# Autodesk Inventor assembly: Robot Assembly
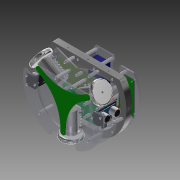
[picture p0: Inventor's stored thumbnail of the model, 180x180]
Saved by Autodesk Inventor 2015 (Build 190159000, 159)
## iProperties
Created: 2016-02-17
Part Number: Robot Assembly
Document SubType Name: Assembly
Designer: 23902
Author: 23902
## Documents named in this file (31)
- C:\Users\James Yelland\git\Work\Design\3D Printing\Version 4\Robot Assembly.iam
- C:\Users\James Yelland\git\Work\Design\3D Printing\Version 4\Motor Mount Plate.ipt
- C:\Users\James Yelland\git\Work\Design\3D Printing\Motor Mount Bracket.ipt
- C:\Users\James Yelland\git\Work\Design\3D Printing\Motor.ipt
- C:\Users\James Yelland\git\Work\Design\3D Printing\Wheel.ipt
- C:\Users\James Yelland\git\Work\Design\3D Printing\Version 4\Middle Plate.ipt
- C:\Users\James Yelland\git\Work\Design\3D Printing\Version 4\Standoff 20.ipt
- C:\Users\James Yelland\git\Work\Design\3D Printing\Version 4\Light Sensor Plate.ipt
- C:\Users\James Yelland\git\Work\Design\3D Printing\Version 4\Light Sensor PCB.ipt
- C:\Users\James Yelland\git\Work\Design\3D Printing\Version 4\Standoff 10.ipt
- C:\Users\James Yelland\git\Work\Design\3D Printing\ArduinoMEGA2560.ipt
- C:\Users\James Yelland\git\Work\Design\3D Printing\Version 4\Standoff 30.ipt
- C:\Users\James Yelland\git\Work\Design\3D Printing\Version 4\Veroboard.ipt
- C:\Users\James Yelland\git\Work\Design\3D Printing\Version 4\M3x20 Screw Nylon.ipt
- C:\Users\James Yelland\git\Work\Design\3D Printing\Version 4\M3x10 Screw Nylon.ipt
- C:\Users\James Yelland\git\Work\Design\3D Printing\Version 4\M3x6 Screw Nylon.ipt
- C:\Users\James Yelland\git\Work\Design\3D Printing\Version 4\M3 Nut Nylon.ipt
- C:\Users\James Yelland\git\Work\Design\3D Printing\Version 4\M3x10 Screw Steel.ipt
- C:\Users\James Yelland\git\Work\Design\3D Printing\Version 4\M3 Nut Steel.ipt
- C:\Users\James Yelland\git\Work\Design\3D Printing\HC-SR04 Sonar.ipt
- C:\Users\James Yelland\git\Work\Design\3D Printing\Version 4\Sonar Mount.ipt
- C:\Users\James Yelland\git\Work\Design\3D Printing\Version 4\M2x10 Screw Steel.ipt
- C:\Users\James Yelland\git\Work\Design\3D Printing\Version 4\M2 Nut Steel.ipt
- C:\Users\James Yelland\git\Work\Design\3D Printing\lcd05-16x2.ipt
- C:\Users\James Yelland\git\Work\Design\3D Printing\Version 4\LCD Plate.ipt
- C:\Users\James Yelland\git\Work\Design\3D Printing\Version 4\Top Plate.ipt
- C:\Users\James Yelland\git\Work\Design\3D Printing\Version 4\Battery.ipt
- C:\Users\James Yelland\git\Work\Design\3D Printing\Version 4\Switch Nut.ipt
- C:\Users\James Yelland\git\Work\Design\3D Printing\Version 4\Switch.ipt
- C:\Users\James Yelland\git\Work\Design\3D Printing\Version 4\Standoff 40.ipt
- C:\Users\James Yelland\git\Work\Design\3D Printing\Compass.ipt
## Components (161 placed, 30 different names)
1. Motor Mount Plate:1 — Mate:1, Mate:2, Mate:3, Mate:22, Mate:23, Mate:24, Mate:25, Mate:26, Mate:27, Mate:28, Mate:29, Mate:30, Mate:31, Mate:32, Mate:33, Mate:34, Mate:35, Mate:101, Mate:102, Mate:103, Mate:104, Mate:113, Mate:114, Mate:115, Mate:116, Mate:117, Mate:118, Mate:127, Mate:128, Mate:129, Mate:130, Mate:131, Mate:132, Mate:155, Mate:156, Mate:157, Mate:158, Mate:159, Mate:160, Mate:161, Mate:162, Mate:182, Mate:183, Mate:184, Mate:185, Mate:186, Mate:187, Mate:203, Mate:204, Mate:205, Mate:206, Mate:207, Mate:208, Mate:209, Mate:210, Mate:211, Mate:212, Mate:213, Mate:214, Mate:223, Mate:224, Mate:225, Mate:226, Mate:227, Mate:228, Mate:229, Mate:230, Mate:249, Mate:250, Mate:251, Mate:252, Mate:253, Mate:254, Mate:255, Mate:256, Mate:257, Mate:269, Mate:270, Mate:272, Mate:274, Mate:278, Mate:280, Mate:281, Mate:282, Mate:284, Mate:288, Mate:289, Mate:290, Mate:291, Mate:293, Mate:294, Mate:295, Mate:296, Mate:297, Mate:298, Mate:299, Mate:300, Mate:301, Mate:302, Mate:303
2. Motor Mount Bracket:1 — Mate:1, Mate:11, Mate:14, Mate:15, Mate:24, Mate:25, Mate:275, Mate:276, Mate:286, Mate:287
3. Motor:1 — Mate:10, Mate:16, Mate:17, Mate:21, Flush:3
4. Wheel:1 — Mate:19, Flush:1
5. Motor Mount Bracket:2 — Mate:2, Mate:10, Mate:16, Mate:17, Mate:22, Mate:23, Mate:267, Mate:268, Mate:277, Mate:279
6. Motor:2 — Mate:11, Mate:14, Mate:15, Mate:19, Flush:1
7. Wheel:2 — Mate:20, Flush:2
8. Motor Mount Bracket:3 — Mate:3, Mate:12, Mate:13, Mate:18, Mate:26, Mate:27, Mate:271, Mate:273, Mate:283, Mate:285
9. Motor:3 — Mate:12, Mate:13, Mate:18, Mate:20, Flush:2
10. Wheel:3 — Mate:21, Flush:3
11. Middle Plate:1 — Mate:36, Mate:37, Mate:38, Mate:191, Mate:192, Mate:193, Mate:194, Mate:195, Mate:196, Mate:197, Mate:198, Mate:199, Mate:200, Mate:201, Mate:202, Mate:315, Mate:316, Mate:317, Mate:318, Mate:319, Mate:320, Mate:321, Mate:322, Mate:323, Mate:324, Mate:325, Mate:326, Mate:327, Mate:328, Mate:329, Mate:330, Mate:452, Mate:453, Mate:454, Mate:455, Mate:462, Mate:463, Mate:464, Mate:465
12. Standoff 20:1 — Mate:28, Mate:33, Mate:38
13. Standoff 20:2 — Mate:29, Mate:35, Mate:36
14. Standoff 20:3 — Mate:31, Mate:32
15. Standoff 20:4 — Mate:30, Mate:34, Mate:37
16. Light Sensor Plate:1 — Mate:152, Mate:153, Mate:154, Mate:163, Mate:164, Mate:165, Mate:215, Mate:216, Mate:217, Mate:218, Mate:219, Mate:220, Mate:221, Mate:222, Mate:362, Mate:384, Mate:385, Mate:386, Mate:387, Mate:388, Mate:389, Mate:390, Mate:391, Mate:392, Mate:393, Mate:394, Mate:395, Mate:396, Mate:510, Mate:511, Mate:512, Mate:515
17. Light Sensor PCB:1 — Mate:152, Mate:153, Mate:154
18. Standoff 20:5 — Mate:103, Mate:104
19. Standoff 20:6 — Mate:101, Mate:102
20. Standoff 10:1 — Mate:114, Mate:128, Mate:263
21. Standoff 10:2 — Mate:115, Mate:129, Mate:266
22. Standoff 10:3 — Mate:116, Mate:130, Mate:133, Mate:260
23. Standoff 10:4 — Mate:118, Mate:131, Mate:259
24. Standoff 10:5 — Mate:117, Mate:126, Mate:132, Mate:261
25. Standoff 10:6 — Mate:113, Mate:125, Mate:127, Mate:265
26. -  -:1 — Mate:125, Mate:126, Mate:133, Mate:234, Mate:235, Mate:236, Mate:237, Mate:238, Mate:239, Mate:240, Mate:241, Mate:242, Mate:243, Mate:244, Mate:245
27. Standoff 30:1 — Mate:157, Mate:162
28. Standoff 30:2 — Mate:159, Mate:161
29. Standoff 30:3 — Mate:155, Mate:156, Mate:163, Mate:164
30. Standoff 30:4 — Mate:158, Mate:160, Mate:165
31. Standoff 10:7 — Mate:182, Mate:186, Mate:190, Mate:258
32. Standoff 10:8 — Mate:183, Mate:187, Mate:188, Mate:189, Mate:262
33. Standoff 10:9 — Mate:184, Mate:185, Mate:264
34. Veroboard:1 — Mate:188, Mate:189, Mate:190, Mate:231, Mate:232, Mate:233, Mate:246, Mate:247, Mate:248
35. M3x20 Screw Nylon:1 — Mate:192, Mate:201
36. M3x20 Screw Nylon:2 — Mate:193, Mate:202
37. M3x20 Screw Nylon:3 — Mate:194, Mate:199
38. M3x20 Screw Nylon:4 — Mate:195, Mate:198
39. M3x20 Screw Nylon:5 — Mate:196, Mate:197
40. M3x20 Screw Nylon:6 — Mate:191, Mate:200
41. M3x10 Screw Nylon:1 — Mate:208, Mate:209
42. M3x10 Screw Nylon:2 — Mate:207, Mate:210
43. M3x10 Screw Nylon:3 — Mate:206, Mate:211
44. M3x10 Screw Nylon:4 — Mate:205, Mate:212
45. M3x10 Screw Nylon:5 — Mate:204, Mate:213
46. M3x10 Screw Nylon:6 — Mate:203, Mate:214
47. M3x10 Screw Nylon:7 — Mate:215, Mate:219
48. M3x10 Screw Nylon:8 — Mate:216, Mate:220
49. M3x10 Screw Nylon:9 — Mate:224, Mate:225
50. M3x10 Screw Nylon:10 — Mate:218, Mate:222
51. M3x10 Screw Nylon:11 — Mate:217, Mate:221
52. M3x10 Screw Nylon:12 — Mate:228, Mate:229
53. M3x10 Screw Nylon:13 — Mate:227, Mate:230
54. M3x10 Screw Nylon:14 — Mate:223, Mate:226
55. M3x6 Screw Nylon:1 — Mate:231, Mate:246
56. M3x6 Screw Nylon:2 — Mate:235, Mate:240
57. M3x6 Screw Nylon:3 — Mate:236, Mate:242
58. M3x6 Screw Nylon:4 — Mate:237, Mate:245
59. M3x6 Screw Nylon:5 — Mate:239, Mate:244
60. M3x6 Screw Nylon:6 — Mate:238, Mate:241
61. M3x6 Screw Nylon:7 — Mate:232, Mate:247
62. M3x6 Screw Nylon:8 — Mate:234, Mate:243
63. M3x6 Screw Nylon:9 — Mate:233, Mate:248
64. M3 Nut Nylon:1 — Mate:253, Mate:260
65. M3 Nut Nylon:2 — Mate:252, Mate:258
66. M3 Nut Nylon:3 — Mate:254, Mate:262
67. M3 Nut Nylon:4 — Mate:255, Mate:261
68. M3 Nut Nylon:5 — Mate:257, Mate:266
69. M3 Nut Nylon:6 — Mate:256, Mate:264
70. M3 Nut Nylon:7 — Mate:251, Mate:259
71. M3 Nut Nylon:8 — Mate:250, Mate:265
72. M3 Nut Nylon:9 — Mate:249, Mate:263
73. M3x10 Screw Steel:1 — Mate:271, Mate:272, Mate:292
74. M3x10 Screw Steel:2 — Mate:273, Mate:274, Mate:310
75. M3x10 Screw Steel:3 — Mate:268, Mate:269, Mate:307
76. M3x10 Screw Steel:4 — Mate:267, Mate:270, Mate:306
77. M3x10 Screw Steel:5 — Mate:283, Mate:284, Mate:308
78. M3x10 Screw Steel:6 — Mate:279, Mate:280, Mate:304
79. M3x10 Screw Steel:7 — Mate:277, Mate:278, Mate:305
80. M3x10 Screw Steel:8 — Mate:275, Mate:282, Mate:311
81. M3x10 Screw Steel:9 — Mate:287, Mate:288, Mate:314
82. M3x10 Screw Steel:10 — Mate:286, Mate:289, Mate:312
83. M3x10 Screw Steel:11 — Mate:285, Mate:290, Mate:309
84. M3x10 Screw Steel:12 — Mate:276, Mate:281, Mate:313
85. M3 Nut Steel:1 — Mate:295, Mate:314
86. M3 Nut Steel:2 — Mate:291, Mate:292
87. M3 Nut Steel:3 — Mate:294, Mate:312
88. M3 Nut Steel:4 — Mate:296, Mate:311
89. M3 Nut Steel:5 — Mate:298, Mate:310
90. M3 Nut Steel:6 — Mate:297, Mate:304
91. M3 Nut Steel:7 — Mate:300, Mate:305
92. M3 Nut Steel:8 — Mate:299, Mate:308
93. M3 Nut Steel:9 — Mate:301, Mate:306
94. M3 Nut Steel:10 — Mate:302, Mate:309
95. M3 Nut Steel:11 — Mate:293, Mate:313
96. M3 Nut Steel:12 — Mate:303, Mate:307
97. Standoff 30:5 — Mate:315, Mate:321
98. Standoff 30:6 — Mate:316, Mate:322
99. Standoff 30:7 — Mate:317, Mate:320, Mate:473, Mate:474
100. Standoff 30:8 — Mate:318, Mate:319, Mate:475
101. M3x20 Screw Nylon:7 — Mate:323, Mate:330
102. M3x20 Screw Nylon:8 — Mate:326, Mate:328
103. M3x20 Screw Nylon:9 — Mate:325, Mate:327
104. M3x20 Screw Nylon:10 — Mate:324, Mate:329
105. HC-SR04 Sonar:1 — Mate:360, Mate:376, Mate:377, Mate:380, Mate:381
106. Sonar Mount:1 — Mate:360, Mate:361, Mate:362, Mate:384, Mate:385, Mate:408, Mate:410, Mate:383, Mate:508, Mate:516
107. M2x10 Screw Steel:1 — Mate:376, Mate:377, Mate:379, Mate:361
108. M2 Nut Steel:1 — Mate:379
109. M2 Nut Steel:2 — Mate:508, Mate:509
110. M2x10 Screw Steel:2 — Mate:380, Mate:381, Mate:383, Mate:509
111. HC-SR04 Sonar:2 — Mate:397, Mate:398, Mate:399, Mate:400, Mate:401, Mate:404, Mate:405
112. Sonar Mount:2 — Mate:386, Mate:387, Mate:388, Mate:397, Mate:398, Mate:399, Mate:402, Mate:403, Mate:412, Mate:414, Mate:513
113. M3x10 Screw Nylon:24 — Mate:394, Mate:396, Mate:409
114. M3x10 Screw Nylon:25 — Mate:393, Mate:395, Mate:411
115. M3x10 Screw Nylon:26 — Mate:389, Mate:390, Mate:413
116. M3x10 Screw Nylon:27 — Mate:391, Mate:392, Mate:415
117. M2 Nut Steel:3 — Mate:403, Mate:406
118. M2x10 Screw Steel:3 — Mate:400, Mate:404, Mate:407
119. M2 Nut Steel:4 — Mate:402, Mate:407
120. M2x10 Screw Steel:4 — Mate:401, Mate:405, Mate:406
121. M3 Nut Nylon:10 — Mate:408, Mate:409
122. M3 Nut Nylon:11 — Mate:410, Mate:411
123. M3 Nut Nylon:12 — Mate:414, Mate:415
124. M3 Nut Nylon:13 — Mate:412, Mate:413
125. Standoff 20:7 — Mate:453, Mate:454, Mate:456, Mate:457
126. Standoff 20:8 — Mate:452, Mate:455, Mate:458
127. LCD Plate:1 — Mate:456, Mate:457, Mate:458, Mate:466, Mate:467, Mate:468, Mate:469, Mate:470, Mate:471, Mate:472, Mate:518, Mate:519, Mate:520, Mate:521, Mate:522, Mate:523, Mate:524, Mate:525
128. M3x20 Screw Nylon:11 — Mate:462, Mate:463
129. M3x20 Screw Nylon:12 — Mate:464, Mate:465
130. M3x10 Screw Nylon:36 — Mate:468, Mate:469
131. M3x10 Screw Nylon:37 — Mate:466, Mate:467
132. lcd05-16x2:1 — Mate:470, Mate:471, Mate:472, Mate:526, Mate:527, Mate:528, Mate:529
133. Top Plate:1 — Mate:473, Mate:474, Mate:475, Mate:476, Mate:477, Mate:478, Mate:479, Mate:480, Mate:481, Mate:482, Mate:483, Mate:484, Mate:485, Mate:486, Mate:487, Mate:488, Mate:489, Mate:490, Mate:491, Mate:492, Mate:493, Mate:494, Mate:495, Flush:4, Flush:5, Mate:496, Mate:497, Mate:507, Flush:6, Flush:7
134. M3x10 Screw Nylon:38 — Mate:489, Mate:491
135. M3x10 Screw Nylon:39 — Mate:503, Mate:504
136. M3x10 Screw Nylon:40 — Mate:488, Mate:490
137. M3x10 Screw Nylon:41 — Mate:505, Mate:506
138. Battery:1 — Mate:507, Flush:6, Flush:7
139. Switch Nut:1 — Mate:496, Mate:499
140. Switch:1 — Mate:492, Mate:495, Flush:5, Mate:499
141. Switch Nut:2 — Mate:497, Mate:498
142. Switch:2 — Mate:493, Mate:494, Flush:4, Mate:498
143. Standoff 40:1 — Mate:477, Mate:487, Mate:500, Mate:501
144. Standoff 40:2 — Mate:476, Mate:486, Mate:502
145. M3x10 Screw Nylon:42 — Mate:480, Mate:482
146. M3x10 Screw Nylon:43 — Mate:478, Mate:484
147. M3x10 Screw Nylon:44 — Mate:481, Mate:483
148. M3x10 Screw Nylon:45 — Mate:479, Mate:485
149. Compass:1 — Mate:500, Mate:501, Mate:502, Mate:503, Mate:504, Mate:505, Mate:506
150. M3x10 Screw Nylon:46 — Mate:511, Mate:515, Mate:517
151. M3x10 Screw Nylon:47 — Mate:510, Mate:512, Mate:514
152. M3 Nut Steel:14 — Mate:513, Mate:514
153. M3 Nut Nylon:14 — Mate:516, Mate:517
154. M2x10 Screw Steel:5 — Mate:524, Mate:525, Mate:530
155. M2x10 Screw Steel:6 — Mate:522, Mate:523, Mate:533
156. M2x10 Screw Steel:7 — Mate:520, Mate:521, Mate:532
157. M2x10 Screw Steel:8 — Mate:518, Mate:519, Mate:531
158. M2 Nut Steel:5 — Mate:529, Mate:533
159. M2 Nut Steel:6 — Mate:528, Mate:532
160. M2 Nut Steel:7 — Mate:527, Mate:531
161. M2 Nut Steel:8 — Mate:526, Mate:530
## Relationships (341: Mate 334, Flush 7)
- Mate:1: Motor Mount Plate:1 ↔ Motor Mount Bracket:1
- Mate:2: Motor Mount Plate:1 ↔ Motor Mount Bracket:2
- Mate:3: Motor Mount Plate:1 ↔ Motor Mount Bracket:3
- Mate:10: Motor:1 ↔ Motor Mount Bracket:2
- Mate:11: Motor Mount Bracket:1 ↔ Motor:2
- Mate:12: Motor Mount Bracket:3 ↔ Motor:3
- Mate:13: Motor Mount Bracket:3 ↔ Motor:3
- Mate:14: Motor Mount Bracket:1 ↔ Motor:2
- Mate:15: Motor Mount Bracket:1 ↔ Motor:2
- Mate:16: Motor:1 ↔ Motor Mount Bracket:2
- Mate:17: Motor:1 ↔ Motor Mount Bracket:2
- Mate:18: Motor Mount Bracket:3 ↔ Motor:3
- Mate:19: Wheel:1 ↔ Motor:2
- Flush:1: Wheel:1 ↔ Motor:2
- Mate:20: Wheel:2 ↔ Motor:3
- Flush:2: Wheel:2 ↔ Motor:3
- Mate:21: Motor:1 ↔ Wheel:3
- Flush:3: Motor:1 ↔ Wheel:3
- Mate:22: Motor Mount Plate:1 ↔ Motor Mount Bracket:2
- Mate:23: Motor Mount Plate:1 ↔ Motor Mount Bracket:2
- Mate:24: Motor Mount Plate:1 ↔ Motor Mount Bracket:1
- Mate:25: Motor Mount Plate:1 ↔ Motor Mount Bracket:1
- Mate:26: Motor Mount Plate:1 ↔ Motor Mount Bracket:3
- Mate:27: Motor Mount Plate:1 ↔ Motor Mount Bracket:3
- Mate:28: Motor Mount Plate:1 ↔ Standoff 20:1
- Mate:29: Motor Mount Plate:1 ↔ Standoff 20:2
- Mate:30: Motor Mount Plate:1 ↔ Standoff 20:4
- Mate:31: Motor Mount Plate:1 ↔ Standoff 20:3
- Mate:32: Motor Mount Plate:1 ↔ Standoff 20:3
- Mate:33: Motor Mount Plate:1 ↔ Standoff 20:1
- Mate:34: Motor Mount Plate:1 ↔ Standoff 20:4
- Mate:35: Motor Mount Plate:1 ↔ Standoff 20:2
- Mate:36: Middle Plate:1 ↔ Standoff 20:2
- Mate:37: Middle Plate:1 ↔ Standoff 20:4
- Mate:38: Middle Plate:1 ↔ Standoff 20:1
- Mate:101: Motor Mount Plate:1 ↔ Standoff 20:6
- Mate:102: Motor Mount Plate:1 ↔ Standoff 20:6
- Mate:103: Motor Mount Plate:1 ↔ Standoff 20:5
- Mate:104: Motor Mount Plate:1 ↔ Standoff 20:5
- Mate:113: Motor Mount Plate:1 ↔ Standoff 10:6
- Mate:114: Motor Mount Plate:1 ↔ Standoff 10:1
- Mate:115: Motor Mount Plate:1 ↔ Standoff 10:2
- Mate:116: Motor Mount Plate:1 ↔ Standoff 10:3
- Mate:117: Motor Mount Plate:1 ↔ Standoff 10:5
- Mate:118: Motor Mount Plate:1 ↔ Standoff 10:4
- Mate:125: Standoff 10:6 ↔ -  -:1
- Mate:126: Standoff 10:5 ↔ -  -:1
- Mate:127: Motor Mount Plate:1 ↔ Standoff 10:6
- Mate:128: Motor Mount Plate:1 ↔ Standoff 10:1
- Mate:129: Motor Mount Plate:1 ↔ Standoff 10:2
- Mate:130: Motor Mount Plate:1 ↔ Standoff 10:3
- Mate:131: Motor Mount Plate:1 ↔ Standoff 10:4
- Mate:132: Motor Mount Plate:1 ↔ Standoff 10:5
- Mate:133: Standoff 10:3 ↔ -  -:1
- Mate:152: Light Sensor Plate:1 ↔ Light Sensor PCB:1
- Mate:153: Light Sensor Plate:1 ↔ Light Sensor PCB:1
- Mate:154: Light Sensor Plate:1 ↔ Light Sensor PCB:1
- Mate:155: Motor Mount Plate:1 ↔ Standoff 30:3
- Mate:156: Motor Mount Plate:1 ↔ Standoff 30:3
- Mate:157: Motor Mount Plate:1 ↔ Standoff 30:1
- Mate:158: Motor Mount Plate:1 ↔ Standoff 30:4
- Mate:159: Motor Mount Plate:1 ↔ Standoff 30:2
- Mate:160: Motor Mount Plate:1 ↔ Standoff 30:4
- Mate:161: Motor Mount Plate:1 ↔ Standoff 30:2
- Mate:162: Motor Mount Plate:1 ↔ Standoff 30:1
- Mate:163: Light Sensor Plate:1 ↔ Standoff 30:3
- Mate:164: Light Sensor Plate:1 ↔ Standoff 30:3
- Mate:165: Light Sensor Plate:1 ↔ Standoff 30:4
- Mate:182: Motor Mount Plate:1 ↔ Standoff 10:7
- Mate:183: Motor Mount Plate:1 ↔ Standoff 10:8
- Mate:184: Motor Mount Plate:1 ↔ Standoff 10:9
- Mate:185: Motor Mount Plate:1 ↔ Standoff 10:9
- Mate:186: Motor Mount Plate:1 ↔ Standoff 10:7
- Mate:187: Motor Mount Plate:1 ↔ Standoff 10:8
- Mate:188: Standoff 10:8 ↔ Veroboard:1
- Mate:189: Standoff 10:8 ↔ Veroboard:1
- Mate:190: Standoff 10:7 ↔ Veroboard:1
- Mate:191: Middle Plate:1 ↔ M3x20 Screw Nylon:6
- Mate:192: Middle Plate:1 ↔ M3x20 Screw Nylon:1
- Mate:193: Middle Plate:1 ↔ M3x20 Screw Nylon:2
- Mate:194: Middle Plate:1 ↔ M3x20 Screw Nylon:3
- Mate:195: Middle Plate:1 ↔ M3x20 Screw Nylon:4
- Mate:196: Middle Plate:1 ↔ M3x20 Screw Nylon:5
- Mate:197: Middle Plate:1 ↔ M3x20 Screw Nylon:5
- Mate:198: Middle Plate:1 ↔ M3x20 Screw Nylon:4
- Mate:199: Middle Plate:1 ↔ M3x20 Screw Nylon:3
- Mate:200: Middle Plate:1 ↔ M3x20 Screw Nylon:6
- Mate:201: Middle Plate:1 ↔ M3x20 Screw Nylon:1
- Mate:202: Middle Plate:1 ↔ M3x20 Screw Nylon:2
- Mate:203: Motor Mount Plate:1 ↔ M3x10 Screw Nylon:6
- Mate:204: Motor Mount Plate:1 ↔ M3x10 Screw Nylon:5
- Mate:205: Motor Mount Plate:1 ↔ M3x10 Screw Nylon:4
- Mate:206: Motor Mount Plate:1 ↔ M3x10 Screw Nylon:3
- Mate:207: Motor Mount Plate:1 ↔ M3x10 Screw Nylon:2
- Mate:208: Motor Mount Plate:1 ↔ M3x10 Screw Nylon:1
- Mate:209: Motor Mount Plate:1 ↔ M3x10 Screw Nylon:1
- Mate:210: Motor Mount Plate:1 ↔ M3x10 Screw Nylon:2
- Mate:211: Motor Mount Plate:1 ↔ M3x10 Screw Nylon:3
- Mate:212: Motor Mount Plate:1 ↔ M3x10 Screw Nylon:4
- Mate:213: Motor Mount Plate:1 ↔ M3x10 Screw Nylon:5
- Mate:214: Motor Mount Plate:1 ↔ M3x10 Screw Nylon:6
- Mate:215: Light Sensor Plate:1 ↔ M3x10 Screw Nylon:7
- Mate:216: Light Sensor Plate:1 ↔ M3x10 Screw Nylon:8
- Mate:217: Light Sensor Plate:1 ↔ M3x10 Screw Nylon:11
- Mate:218: Light Sensor Plate:1 ↔ M3x10 Screw Nylon:10
- Mate:219: Light Sensor Plate:1 ↔ M3x10 Screw Nylon:7
- Mate:220: Light Sensor Plate:1 ↔ M3x10 Screw Nylon:8
- Mate:221: Light Sensor Plate:1 ↔ M3x10 Screw Nylon:11
- Mate:222: Light Sensor Plate:1 ↔ M3x10 Screw Nylon:10
- Mate:223: Motor Mount Plate:1 ↔ M3x10 Screw Nylon:14
- Mate:224: Motor Mount Plate:1 ↔ M3x10 Screw Nylon:9
- Mate:225: Motor Mount Plate:1 ↔ M3x10 Screw Nylon:9
- Mate:226: Motor Mount Plate:1 ↔ M3x10 Screw Nylon:14
- Mate:227: Motor Mount Plate:1 ↔ M3x10 Screw Nylon:13
- Mate:228: Motor Mount Plate:1 ↔ M3x10 Screw Nylon:12
- Mate:229: Motor Mount Plate:1 ↔ M3x10 Screw Nylon:12
- Mate:230: Motor Mount Plate:1 ↔ M3x10 Screw Nylon:13
- Mate:231: Veroboard:1 ↔ M3x6 Screw Nylon:1
- Mate:232: Veroboard:1 ↔ M3x6 Screw Nylon:7
- Mate:233: Veroboard:1 ↔ M3x6 Screw Nylon:9
- Mate:234: -  -:1 ↔ M3x6 Screw Nylon:8
- Mate:235: -  -:1 ↔ M3x6 Screw Nylon:2
- Mate:236: -  -:1 ↔ M3x6 Screw Nylon:3
- Mate:237: -  -:1 ↔ M3x6 Screw Nylon:4
- Mate:238: -  -:1 ↔ M3x6 Screw Nylon:6
- Mate:239: -  -:1 ↔ M3x6 Screw Nylon:5
- Mate:240: -  -:1 ↔ M3x6 Screw Nylon:2
- Mate:241: -  -:1 ↔ M3x6 Screw Nylon:6
- Mate:242: -  -:1 ↔ M3x6 Screw Nylon:3
- Mate:243: -  -:1 ↔ M3x6 Screw Nylon:8
- Mate:244: -  -:1 ↔ M3x6 Screw Nylon:5
- Mate:245: -  -:1 ↔ M3x6 Screw Nylon:4
- Mate:246: Veroboard:1 ↔ M3x6 Screw Nylon:1
- Mate:247: Veroboard:1 ↔ M3x6 Screw Nylon:7
- Mate:248: Veroboard:1 ↔ M3x6 Screw Nylon:9
- Mate:249: Motor Mount Plate:1 ↔ M3 Nut Nylon:9
- Mate:250: Motor Mount Plate:1 ↔ M3 Nut Nylon:8
- Mate:251: Motor Mount Plate:1 ↔ M3 Nut Nylon:7
- Mate:252: Motor Mount Plate:1 ↔ M3 Nut Nylon:2
- Mate:253: Motor Mount Plate:1 ↔ M3 Nut Nylon:1
- Mate:254: Motor Mount Plate:1 ↔ M3 Nut Nylon:3
- Mate:255: Motor Mount Plate:1 ↔ M3 Nut Nylon:4
- Mate:256: Motor Mount Plate:1 ↔ M3 Nut Nylon:6
- Mate:257: Motor Mount Plate:1 ↔ M3 Nut Nylon:5
- Mate:258: Standoff 10:7 ↔ M3 Nut Nylon:2
- Mate:259: Standoff 10:4 ↔ M3 Nut Nylon:7
- Mate:260: Standoff 10:3 ↔ M3 Nut Nylon:1
- Mate:261: Standoff 10:5 ↔ M3 Nut Nylon:4
- Mate:262: Standoff 10:8 ↔ M3 Nut Nylon:3
- Mate:263: Standoff 10:1 ↔ M3 Nut Nylon:9
- Mate:264: Standoff 10:9 ↔ M3 Nut Nylon:6
- Mate:265: Standoff 10:6 ↔ M3 Nut Nylon:8
- Mate:266: Standoff 10:2 ↔ M3 Nut Nylon:5
- Mate:267: Motor Mount Bracket:2 ↔ M3x10 Screw Steel:4
- Mate:268: Motor Mount Bracket:2 ↔ M3x10 Screw Steel:3
- Mate:269: Motor Mount Plate:1 ↔ M3x10 Screw Steel:3
- Mate:270: Motor Mount Plate:1 ↔ M3x10 Screw Steel:4
- Mate:271: Motor Mount Bracket:3 ↔ M3x10 Screw Steel:1
- Mate:272: Motor Mount Plate:1 ↔ M3x10 Screw Steel:1
- Mate:273: Motor Mount Bracket:3 ↔ M3x10 Screw Steel:2
- Mate:274: Motor Mount Plate:1 ↔ M3x10 Screw Steel:2
- Mate:275: Motor Mount Bracket:1 ↔ M3x10 Screw Steel:8
- Mate:276: Motor Mount Bracket:1 ↔ M3x10 Screw Steel:12
- Mate:277: Motor Mount Bracket:2 ↔ M3x10 Screw Steel:7
- Mate:278: Motor Mount Plate:1 ↔ M3x10 Screw Steel:7
- Mate:279: Motor Mount Bracket:2 ↔ M3x10 Screw Steel:6
- Mate:280: Motor Mount Plate:1 ↔ M3x10 Screw Steel:6
- Mate:281: Motor Mount Plate:1 ↔ M3x10 Screw Steel:12
- Mate:282: Motor Mount Plate:1 ↔ M3x10 Screw Steel:8
- Mate:283: Motor Mount Bracket:3 ↔ M3x10 Screw Steel:5
- Mate:284: Motor Mount Plate:1 ↔ M3x10 Screw Steel:5
- Mate:285: Motor Mount Bracket:3 ↔ M3x10 Screw Steel:11
- Mate:286: Motor Mount Bracket:1 ↔ M3x10 Screw Steel:10
- Mate:287: Motor Mount Bracket:1 ↔ M3x10 Screw Steel:9
- Mate:288: Motor Mount Plate:1 ↔ M3x10 Screw Steel:9
- Mate:289: Motor Mount Plate:1 ↔ M3x10 Screw Steel:10
- Mate:290: Motor Mount Plate:1 ↔ M3x10 Screw Steel:11
- Mate:291: Motor Mount Plate:1 ↔ M3 Nut Steel:2
- Mate:292: M3x10 Screw Steel:1 ↔ M3 Nut Steel:2
- Mate:293: Motor Mount Plate:1 ↔ M3 Nut Steel:11
- Mate:294: Motor Mount Plate:1 ↔ M3 Nut Steel:3
- Mate:295: Motor Mount Plate:1 ↔ M3 Nut Steel:1
- Mate:296: Motor Mount Plate:1 ↔ M3 Nut Steel:4
- Mate:297: Motor Mount Plate:1 ↔ M3 Nut Steel:6
- Mate:298: Motor Mount Plate:1 ↔ M3 Nut Steel:5
- Mate:299: Motor Mount Plate:1 ↔ M3 Nut Steel:8
- Mate:300: Motor Mount Plate:1 ↔ M3 Nut Steel:7
- Mate:301: Motor Mount Plate:1 ↔ M3 Nut Steel:9
- Mate:302: Motor Mount Plate:1 ↔ M3 Nut Steel:10
- Mate:303: Motor Mount Plate:1 ↔ M3 Nut Steel:12
- Mate:304: M3x10 Screw Steel:6 ↔ M3 Nut Steel:6
- Mate:305: M3x10 Screw Steel:7 ↔ M3 Nut Steel:7
- Mate:306: M3x10 Screw Steel:4 ↔ M3 Nut Steel:9
- Mate:307: M3x10 Screw Steel:3 ↔ M3 Nut Steel:12
- Mate:308: M3x10 Screw Steel:5 ↔ M3 Nut Steel:8
- Mate:309: M3x10 Screw Steel:11 ↔ M3 Nut Steel:10
- Mate:310: M3x10 Screw Steel:2 ↔ M3 Nut Steel:5
- Mate:311: M3x10 Screw Steel:8 ↔ M3 Nut Steel:4
- Mate:312: M3x10 Screw Steel:10 ↔ M3 Nut Steel:3
- Mate:313: M3x10 Screw Steel:12 ↔ M3 Nut Steel:11
- Mate:314: M3x10 Screw Steel:9 ↔ M3 Nut Steel:1
- Mate:315: Middle Plate:1 ↔ Standoff 30:5
- Mate:316: Middle Plate:1 ↔ Standoff 30:6
- Mate:317: Middle Plate:1 ↔ Standoff 30:7
- Mate:318: Middle Plate:1 ↔ Standoff 30:8
- Mate:319: Middle Plate:1 ↔ Standoff 30:8
- Mate:320: Middle Plate:1 ↔ Standoff 30:7
- Mate:321: Middle Plate:1 ↔ Standoff 30:5
- Mate:322: Middle Plate:1 ↔ Standoff 30:6
- Mate:323: Middle Plate:1 ↔ M3x20 Screw Nylon:7
- Mate:324: Middle Plate:1 ↔ M3x20 Screw Nylon:10
- Mate:325: Middle Plate:1 ↔ M3x20 Screw Nylon:9
- Mate:326: Middle Plate:1 ↔ M3x20 Screw Nylon:8
- Mate:327: Middle Plate:1 ↔ M3x20 Screw Nylon:9
- Mate:328: Middle Plate:1 ↔ M3x20 Screw Nylon:8
- Mate:329: Middle Plate:1 ↔ M3x20 Screw Nylon:10
- Mate:330: Middle Plate:1 ↔ M3x20 Screw Nylon:7
- Mate:360 (1 mm): HC-SR04 Sonar:1 ↔ Sonar Mount:1
- Mate:361: Sonar Mount:1 ↔ M2x10 Screw Steel:1
- Mate:362: Light Sensor Plate:1 ↔ Sonar Mount:1
- Mate:376: HC-SR04 Sonar:1 ↔ M2x10 Screw Steel:1
- Mate:377: HC-SR04 Sonar:1 ↔ M2x10 Screw Steel:1
- Mate:379: M2x10 Screw Steel:1 ↔ M2 Nut Steel:1
- Mate:380: HC-SR04 Sonar:1 ↔ M2x10 Screw Steel:2
- Mate:381: HC-SR04 Sonar:1 ↔ M2x10 Screw Steel:2
- Mate:383: Sonar Mount:1 ↔ M2x10 Screw Steel:2
- Mate:384: Light Sensor Plate:1 ↔ Sonar Mount:1
- Mate:385: Light Sensor Plate:1 ↔ Sonar Mount:1
- Mate:386: Light Sensor Plate:1 ↔ Sonar Mount:2
- Mate:387: Light Sensor Plate:1 ↔ Sonar Mount:2
- Mate:388: Light Sensor Plate:1 ↔ Sonar Mount:2
- Mate:389: Light Sensor Plate:1 ↔ M3x10 Screw Nylon:26
- Mate:390: Light Sensor Plate:1 ↔ M3x10 Screw Nylon:26
- Mate:391: Light Sensor Plate:1 ↔ M3x10 Screw Nylon:27
- Mate:392: Light Sensor Plate:1 ↔ M3x10 Screw Nylon:27
- Mate:393: Light Sensor Plate:1 ↔ M3x10 Screw Nylon:25
- Mate:394: Light Sensor Plate:1 ↔ M3x10 Screw Nylon:24
- Mate:395: Light Sensor Plate:1 ↔ M3x10 Screw Nylon:25
- Mate:396: Light Sensor Plate:1 ↔ M3x10 Screw Nylon:24
- Mate:397 (1 mm): HC-SR04 Sonar:2 ↔ Sonar Mount:2
- Mate:398: HC-SR04 Sonar:2 ↔ Sonar Mount:2
- Mate:399: HC-SR04 Sonar:2 ↔ Sonar Mount:2
- Mate:400: HC-SR04 Sonar:2 ↔ M2x10 Screw Steel:3
- Mate:401: HC-SR04 Sonar:2 ↔ M2x10 Screw Steel:4
- Mate:402: Sonar Mount:2 ↔ M2 Nut Steel:4
- Mate:403: Sonar Mount:2 ↔ M2 Nut Steel:3
- Mate:404: HC-SR04 Sonar:2 ↔ M2x10 Screw Steel:3
- Mate:405: HC-SR04 Sonar:2 ↔ M2x10 Screw Steel:4
- Mate:406: M2 Nut Steel:3 ↔ M2x10 Screw Steel:4
- Mate:407: M2x10 Screw Steel:3 ↔ M2 Nut Steel:4
- Mate:408: Sonar Mount:1 ↔ M3 Nut Nylon:10
- Mate:409: M3x10 Screw Nylon:24 ↔ M3 Nut Nylon:10
- Mate:410: Sonar Mount:1 ↔ M3 Nut Nylon:11
- Mate:411: M3x10 Screw Nylon:25 ↔ M3 Nut Nylon:11
- Mate:412: Sonar Mount:2 ↔ M3 Nut Nylon:13
- Mate:413: M3x10 Screw Nylon:26 ↔ M3 Nut Nylon:13
- Mate:414: Sonar Mount:2 ↔ M3 Nut Nylon:12
- Mate:415: M3x10 Screw Nylon:27 ↔ M3 Nut Nylon:12
- Mate:452: Middle Plate:1 ↔ Standoff 20:8
- Mate:453: Middle Plate:1 ↔ Standoff 20:7
- Mate:454: Middle Plate:1 ↔ Standoff 20:7
- Mate:455: Middle Plate:1 ↔ Standoff 20:8
- Mate:456: Standoff 20:7 ↔ LCD Plate:1
- Mate:457: Standoff 20:7 ↔ LCD Plate:1
- Mate:458: Standoff 20:8 ↔ LCD Plate:1
- Mate:462: Middle Plate:1 ↔ M3x20 Screw Nylon:11
- Mate:463: Middle Plate:1 ↔ M3x20 Screw Nylon:11
- Mate:464: Middle Plate:1 ↔ M3x20 Screw Nylon:12
- Mate:465: Middle Plate:1 ↔ M3x20 Screw Nylon:12
- Mate:466: LCD Plate:1 ↔ M3x10 Screw Nylon:37
- Mate:467: LCD Plate:1 ↔ M3x10 Screw Nylon:37
- Mate:468: LCD Plate:1 ↔ M3x10 Screw Nylon:36
- Mate:469: LCD Plate:1 ↔ M3x10 Screw Nylon:36
- Mate:470 (3 mm): LCD Plate:1 ↔ lcd05-16x2:1
- Mate:471: LCD Plate:1 ↔ lcd05-16x2:1
- Mate:472: LCD Plate:1 ↔ lcd05-16x2:1
- Mate:473: Standoff 30:7 ↔ Top Plate:1
- Mate:474: Standoff 30:7 ↔ Top Plate:1
- Mate:475: Standoff 30:8 ↔ Top Plate:1
- Mate:476: Top Plate:1 ↔ Standoff 40:2
- Mate:477: Top Plate:1 ↔ Standoff 40:1
- Mate:478: Top Plate:1 ↔ M3x10 Screw Nylon:43
- Mate:479: Top Plate:1 ↔ M3x10 Screw Nylon:45
- Mate:480: Top Plate:1 ↔ M3x10 Screw Nylon:42
- Mate:481: Top Plate:1 ↔ M3x10 Screw Nylon:44
- Mate:482: Top Plate:1 ↔ M3x10 Screw Nylon:42
- Mate:483: Top Plate:1 ↔ M3x10 Screw Nylon:44
- Mate:484: Top Plate:1 ↔ M3x10 Screw Nylon:43
- Mate:485: Top Plate:1 ↔ M3x10 Screw Nylon:45
- Mate:486: Top Plate:1 ↔ Standoff 40:2
- Mate:487: Top Plate:1 ↔ Standoff 40:1
- Mate:488: Top Plate:1 ↔ M3x10 Screw Nylon:40
- Mate:489: Top Plate:1 ↔ M3x10 Screw Nylon:38
- Mate:490: Top Plate:1 ↔ M3x10 Screw Nylon:40
- Mate:491: Top Plate:1 ↔ M3x10 Screw Nylon:38
- Mate:492: Top Plate:1 ↔ Switch:1
- Mate:493: Top Plate:1 ↔ Switch:2
- Mate:494: Top Plate:1 ↔ Switch:2
- Mate:495: Top Plate:1 ↔ Switch:1
- Flush:4 (5.6 mm): Top Plate:1 ↔ Switch:2
- Flush:5 (5.6 mm): Top Plate:1 ↔ Switch:1
- Mate:496: Top Plate:1 ↔ Switch Nut:1
- Mate:497: Top Plate:1 ↔ Switch Nut:2
- Mate:498: Switch Nut:2 ↔ Switch:2
- Mate:499: Switch Nut:1 ↔ Switch:1
- Mate:500: Standoff 40:1 ↔ Compass:1
- Mate:501: Standoff 40:1 ↔ Compass:1
- Mate:502: Standoff 40:2 ↔ Compass:1
- Mate:503: M3x10 Screw Nylon:39 ↔ Compass:1
- Mate:504: M3x10 Screw Nylon:39 ↔ Compass:1
- Mate:505: M3x10 Screw Nylon:41 ↔ Compass:1
- Mate:506: M3x10 Screw Nylon:41 ↔ Compass:1
- Mate:507: Top Plate:1 ↔ Battery:1
- Flush:6 (16 mm): Top Plate:1 ↔ Battery:1
- Flush:7 (3 mm): Top Plate:1 ↔ Battery:1
- Mate:508: Sonar Mount:1 ↔ M2 Nut Steel:2
- Mate:509: M2 Nut Steel:2 ↔ M2x10 Screw Steel:2
- Mate:510: Light Sensor Plate:1 ↔ M3x10 Screw Nylon:47
- Mate:511: Light Sensor Plate:1 ↔ M3x10 Screw Nylon:46
- Mate:512: Light Sensor Plate:1 ↔ M3x10 Screw Nylon:47
- Mate:513: Sonar Mount:2 ↔ M3 Nut Steel:14
- Mate:514: M3x10 Screw Nylon:47 ↔ M3 Nut Steel:14
- Mate:515: Light Sensor Plate:1 ↔ M3x10 Screw Nylon:46
- Mate:516: Sonar Mount:1 ↔ M3 Nut Nylon:14
- Mate:517: M3x10 Screw Nylon:46 ↔ M3 Nut Nylon:14
- Mate:518: LCD Plate:1 ↔ M2x10 Screw Steel:8
- Mate:519: LCD Plate:1 ↔ M2x10 Screw Steel:8
- Mate:520: LCD Plate:1 ↔ M2x10 Screw Steel:7
- Mate:521: LCD Plate:1 ↔ M2x10 Screw Steel:7
- Mate:522: LCD Plate:1 ↔ M2x10 Screw Steel:6
- Mate:523: LCD Plate:1 ↔ M2x10 Screw Steel:6
- Mate:524: LCD Plate:1 ↔ M2x10 Screw Steel:5
- Mate:525: LCD Plate:1 ↔ M2x10 Screw Steel:5
- Mate:526: lcd05-16x2:1 ↔ M2 Nut Steel:8
- Mate:527: lcd05-16x2:1 ↔ M2 Nut Steel:7
- Mate:528: lcd05-16x2:1 ↔ M2 Nut Steel:6
- Mate:529: lcd05-16x2:1 ↔ M2 Nut Steel:5
- Mate:530: M2x10 Screw Steel:5 ↔ M2 Nut Steel:8
- Mate:531: M2x10 Screw Steel:8 ↔ M2 Nut Steel:7
- Mate:532: M2x10 Screw Steel:7 ↔ M2 Nut Steel:6
- Mate:533: M2x10 Screw Steel:6 ↔ M2 Nut Steel:5
